# Autodesk Inventor assembly: Cuello
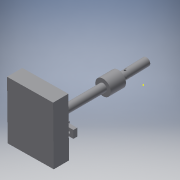
[picture p0: Inventor's stored thumbnail of the model, 180x180]
Saved by Autodesk Inventor 2017 SP1 (Build 210196100, 196)
## iProperties
Part Number: Cuello
Material: Genérico
Document SubType Name: Assembly
Designer: Juan
Author: Juan
## Documents named in this file (4)
- C:\Users\Juan\Documents\Inventor\Cabeza_1\Cuello.iam
- C:\Users\Juan\Documents\Inventor\Cabeza_1\BaseCuello.ipt
- C:\Users\Juan\Documents\Inventor\Cabeza_1\CosaCuello 2.ipt
- C:\Users\Juan\Documents\Inventor\Cabeza_1\CosaCuello.ipt
## Components (3 placed, 3 different names)
1. BaseCuello:1 — De rotación:1
2. CosaCuello 2:1 — De rotación:1, Coincidencia:1
3. CosaCuello:1 — Coincidencia:1
## Relationships (2: RevoluteJoint 1, Mate 1)
- De rotación:1 [RevoluteJoint]: BaseCuello:1 ↔ CosaCuello 2:1
- Coincidencia:1 [Mate]: CosaCuello 2:1 ↔ CosaCuello:1
